# Autodesk Inventor assembly: ZAssembly
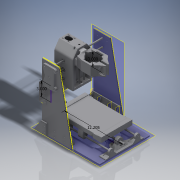
[picture p0: Inventor's stored thumbnail of the model, 180x180]
Saved by Autodesk Inventor 2016 (Build 200138000, 138)
## iProperties
Created: 2016-03-26
Part Number: ZAssembly
Document SubType Name: Assembly
Designer: Scott
Author: Scott
## Documents named in this file (23)
- C:\Users\Scott\Google Drive\Engineering Ideas and Designs\3D printer\Nefarian\ZAssembly.iam
- C:\Users\Scott\Google Drive\Engineering Ideas and Designs\3D printer\Nefarian\Z Nut.ipt
- C:\Users\Scott\Google Drive\Engineering Ideas and Designs\3D printer\Nefarian\ZFrame.ipt
- C:\Users\Scott\Google Drive\Engineering Ideas and Designs\3D printer\Nefarian\Z Slide.ipt
- C:\Users\Scott\Google Drive\Engineering Ideas and Designs\3D printer\Nefarian\Rails.ipt
- C:\Users\Scott\Google Drive\Engineering Ideas and Designs\3D printer\Nefarian\Endstop.ipt
- C:\Users\Scott\Google Drive\Engineering Ideas and Designs\3D printer\Nefarian\Side Walls.ipt
- C:\Users\Scott\Google Drive\Engineering Ideas and Designs\3D printer\Nefarian\BasePlate.ipt
- C:\Users\Scott\Google Drive\Engineering Ideas and Designs\3D printer\Nefarian\Ymotormount.ipt
- C:\Users\Scott\Google Drive\Engineering Ideas and Designs\3D printer\Nefarian\YEnd.ipt
- C:\Users\Scott\Google Drive\Engineering Ideas and Designs\3D printer\Nefarian\Part Plate.ipt
- C:\Users\Scott\Google Drive\Engineering Ideas and Designs\3D printer\Nefarian\EndcapWithSlotholes.ipt
- C:\Users\Scott\Google Drive\Engineering Ideas and Designs\3D printer\Nefarian\YRails.ipt
- C:\Users\Scott\Google Drive\Engineering Ideas and Designs\3D printer\Nefarian\RouterMount.ipt
- C:\Users\Scott\Google Drive\Engineering Ideas and Designs\3D printer\Nefarian\Z Rails.ipt
- C:\Users\Scott\Google Drive\Engineering Ideas and Designs\3D printer\Nefarian\X motor.ipt
- C:\Users\Scott\Google Drive\Engineering Ideas and Designs\3D printer\Nefarian\Back Plate.ipt
- C:\Users\Scott\Google Drive\Engineering Ideas and Designs\3D printer\Nefarian\Backplatemount.ipt
- C:\Users\Scott\Google Drive\Engineering Ideas and Designs\3D printer\Nefarian\Backplatemount_MIR.ipt
- C:\Users\Scott\Google Drive\Engineering Ideas and Designs\3D printer\Nefarian\SidePlateMount.ipt
- C:\Users\Scott\Google Drive\Engineering Ideas and Designs\3D printer\Nefarian\SidePlateMount_MIR.ipt
- C:\Users\Scott\Google Drive\Engineering Ideas and Designs\3D printer\Nefarian\Bed Slide.ipt
- C:\Users\Scott\Google Drive\Engineering Ideas and Designs\3D printer\Nefarian\Bed.ipt
## Components (26 placed, 22 different names)
1. Z Nut:1 — Flush:1, Flush:2, Flush:3, Flush:4, Flush:5, Flush:24, Flush:25, Flush:26, Flush:27
2. ZFrame:1 — Flush:1, Flush:2, Flush:3, Flush:4, Flush:5, Flush:6, Flush:7, Flush:28, Flush:29
3. Z Slide:1 — Flush:6, Flush:7, Flush:8, Flush:9, Flush:10
4. Rails:1 — Flush:9, Flush:10, Mate:1, Mate:2, Mate:3, Mate:4, Mate:6
5. Endstop:1 — Mate:3, Mate:4, Mate:5
6. Endstop:2 — Mate:1, Mate:2, Flush:11, Flush:12
7. Side Walls:1 — Flush:11, Flush:12, Flush:13, Flush:14
8. Side Walls:2 — Mate:5, Mate:6, Flush:30, Flush:31, Flush:32, Flush:33, Flush:38
9. BasePlate:1 — Flush:13, Flush:14, Flush:15, Flush:16, Flush:17, Flush:18, Flush:36, Flush:37
10. Ymotormount:1 — Flush:15, Flush:16, Flush:19, Mate:13, Mate:14, Flush:39
11. YEnd:1 — Flush:17, Flush:18, Flush:22, Flush:23
12. Part Plate:1 — Flush:20, Flush:21, Mate:7, Mate:8, Mate:9, Mate:10, Mate:11, Mate:12
13. EndcapWithSlotholes:1 — Mate:7, Mate:8, Mate:12
14. EndcapWithSlotholes:2 — Mate:9, Mate:10, Mate:11, Flush:40, Flush:41
15. YRails:1 — Flush:22, Flush:23
16. RouterMount:1 — Flush:24, Flush:25, Flush:26, Flush:27
17. Z Rails:1 — Flush:28, Flush:29
18. X motor:1 — Flush:30, Flush:31
19. Back Plate:1 — Flush:32, Flush:33, Flush:34, Flush:35
20. Backplatemount:1 — Flush:34, Flush:35
21. Backplatemount_MIR:1
22. SidePlateMount:1 — Flush:36, Flush:37, Flush:38
23. SidePlateMount_MIR:1
24. X motor:2 — Mate:13, Mate:14, Flush:39
25. Bed Slide:1 — Flush:40, Flush:41, Flush:42
26. Bed:1 — Flush:43, Flush:44
## Relationships (58: Flush 44, Mate 14)
- Flush:1: Z Nut:1 ↔ ZFrame:1
- Flush:2: Z Nut:1 ↔ ZFrame:1
- Flush:3: Z Nut:1 ↔ ZFrame:1
- Flush:4 (3.175 mm): Z Nut:1 ↔ ZFrame:1
- Flush:5: Z Nut:1 ↔ ZFrame:1
- Flush:6: ZFrame:1 ↔ Z Slide:1
- Flush:7: ZFrame:1 ↔ Z Slide:1
- Flush:8 (49.2125 mm): Z Slide:1
- Flush:9: Z Slide:1 ↔ Rails:1
- Flush:10: Z Slide:1 ↔ Rails:1
- Mate:1: Rails:1 ↔ Endstop:2
- Mate:2: Rails:1 ↔ Endstop:2
- Mate:3: Rails:1 ↔ Endstop:1
- Mate:4: Rails:1 ↔ Endstop:1
- Flush:11: Endstop:2 ↔ Side Walls:1
- Flush:12: Endstop:2 ↔ Side Walls:1
- Mate:5: Endstop:1 ↔ Side Walls:2
- Mate:6: Rails:1 ↔ Side Walls:2
- Flush:13: Side Walls:1 ↔ BasePlate:1
- Flush:14: Side Walls:1 ↔ BasePlate:1
- Flush:15: BasePlate:1 ↔ Ymotormount:1
- Flush:16: BasePlate:1 ↔ Ymotormount:1
- Flush:17: BasePlate:1 ↔ YEnd:1
- Flush:18: BasePlate:1 ↔ YEnd:1
- Flush:19 (6.35 mm): Ymotormount:1
- Flush:20: Part Plate:1
- Flush:21: Part Plate:1
- Mate:7: Part Plate:1 ↔ EndcapWithSlotholes:1
- Mate:8: Part Plate:1 ↔ EndcapWithSlotholes:1
- Mate:9: Part Plate:1 ↔ EndcapWithSlotholes:2
- Mate:10: Part Plate:1 ↔ EndcapWithSlotholes:2
- Mate:11: Part Plate:1 ↔ EndcapWithSlotholes:2
- Mate:12: Part Plate:1 ↔ EndcapWithSlotholes:1
- Flush:22: YEnd:1 ↔ YRails:1
- Flush:23: YEnd:1 ↔ YRails:1
- Flush:24: Z Nut:1 ↔ RouterMount:1
- Flush:25: Z Nut:1 ↔ RouterMount:1
- Flush:26: Z Nut:1 ↔ RouterMount:1
- Flush:27: Z Nut:1 ↔ RouterMount:1
- Flush:28: ZFrame:1 ↔ Z Rails:1
- Flush:29: ZFrame:1 ↔ Z Rails:1
- Flush:30: Side Walls:2 ↔ X motor:1
- Flush:31: Side Walls:2 ↔ X motor:1
- Flush:32: Side Walls:2 ↔ Back Plate:1
- Flush:33: Side Walls:2 ↔ Back Plate:1
- Flush:34: Back Plate:1 ↔ Backplatemount:1
- Flush:35: Back Plate:1 ↔ Backplatemount:1
- Flush:36: BasePlate:1 ↔ SidePlateMount:1
- Flush:37: BasePlate:1 ↔ SidePlateMount:1
- Flush:38: Side Walls:2 ↔ SidePlateMount:1
- Mate:13: Ymotormount:1 ↔ X motor:2
- Mate:14: Ymotormount:1 ↔ X motor:2
- Flush:39: Ymotormount:1 ↔ X motor:2
- Flush:40: EndcapWithSlotholes:2 ↔ Bed Slide:1
- Flush:41 (-76.2 mm): EndcapWithSlotholes:2 ↔ Bed Slide:1
- Flush:42 (76.2 mm): Bed Slide:1
- Flush:43: Bed:1
- Flush:44: Bed:1
